# Autodesk Inventor assembly: valve driver
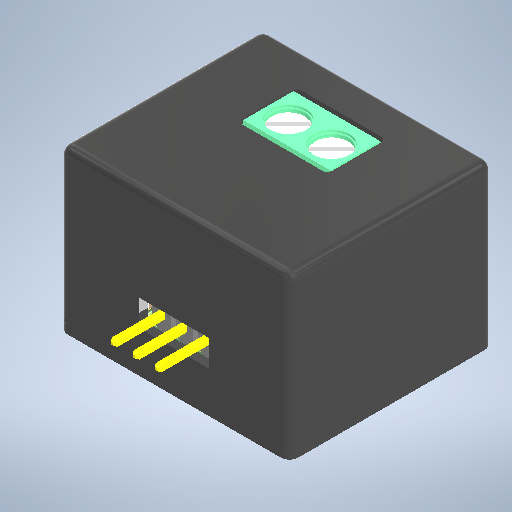
[picture p0: Inventor's stored thumbnail of the model, 512x512]
Saved by Autodesk Inventor 2025.4 (Build 294407000, 407)
## iProperties
Created: 2025-05-14
Part Number: valve driver
Document SubType Name: Assembly
Designer: Yuhsuan Chen
Author: Yuhsuan Chen
## Documents named in this file (4)
- C:\Users\Yuhsuan Chen\Desktop\github\fablabs-valve-driver\mCAD\valve driver master-pin header.iam
- C:\Users\Yuhsuan Chen\Desktop\github\fablabs-valve-driver\mCAD\PCBA\valve_driver.iam
- C:\Users\Yuhsuan Chen\Desktop\github\fablabs-valve-driver\mCAD\bottom cover-pin header.ipt
- C:\Users\Yuhsuan Chen\Desktop\github\fablabs-valve-driver\mCAD\top cover-pin header.ipt
## Components (3 placed, 3 different names)
1. valve_driver:2 [sub-assembly] — Mate:1, Mate:2, Flush:1, Mate:8
2. bottom cover-pin header:1 — Mate:3, Flush:3, Mate:8
3. top cover-pin header:1 — Mate:4, Flush:2
## Relationships (8: Mate 5, Flush 3)
- Mate:1: valve_driver:2
- Mate:2: valve_driver:2
- Flush:1: valve_driver:2
- Mate:3: bottom cover-pin header:1
- Mate:4 (-0.55 mm): top cover-pin header:1
- Flush:2: top cover-pin header:1
- Flush:3: bottom cover-pin header:1
- Mate:8: valve_driver:2 ↔ bottom cover-pin header:1
